# Autodesk Inventor assembly: pinion_assembly
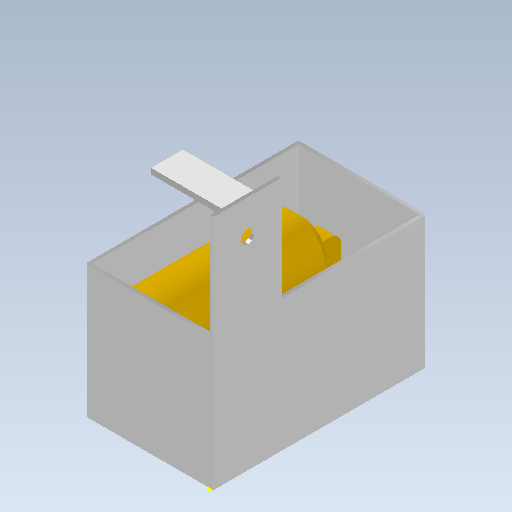
[picture p0: Inventor's stored thumbnail of the model, 512x512]
Saved by Autodesk Inventor 2021 (Build 250183000, 183)
## iProperties
Created: 2021-06-23
Part Number: pinion_assembly
Document SubType Name: Assembly
## Documents named in this file (4)
- C:\Users\ocon0143\OneDrive - Flinders\Advn Mech Design Shared\6_Development\2_Design\inventor\rack_pinion\pinion_assembly.iam
- C:\Users\ocon0143\OneDrive - Flinders\Advn Mech Design Shared\6_Development\2_Design\inventor\support\reel\motor.ipt
- C:\Users\ocon0143\OneDrive - Flinders\Advn Mech Design Shared\6_Development\2_Design\inventor\rack_pinion\rp_box.ipt
- C:\Users\ocon0143\OneDrive - Flinders\Advn Mech Design Shared\6_Development\2_Design\inventor\rack_pinion\support_rp_roof.ipt
## Components (3 placed, 3 different names)
1. motor:1 — Mate:1, Mate:2, Mate:3
2. rp_box:1 — Mate:1, Mate:2, Mate:3, Mate:4, Flush:1, Flush:2
3. support_rp_roof:1 — Mate:4, Flush:1, Flush:2
## Relationships (6: Mate 4, Flush 2)
- Mate:1: motor:1 ↔ rp_box:1
- Mate:2: motor:1 ↔ rp_box:1
- Mate:3: motor:1 ↔ rp_box:1
- Mate:4: rp_box:1 ↔ support_rp_roof:1
- Flush:1: rp_box:1 ↔ support_rp_roof:1
- Flush:2 (10 mm): rp_box:1 ↔ support_rp_roof:1
